# Autodesk Inventor assembly: Magnet
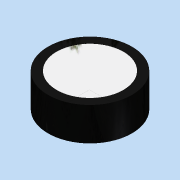
[picture p0: Inventor's stored thumbnail of the model, 180x180]
Saved by Autodesk Inventor 2015 (Build 190159000, 159)
## iProperties
Created: 2015-11-09
Part Number: Magnet
Document SubType Name: Assembly
Designer: Raphael
Author: Raphael
## Documents named in this file (3)
- \\psf\Home\Documents\electric-skateboard\CAD\Magnet.iam
- \\psf\Home\Documents\electric-skateboard\CAD\MagnetHolder.ipt
- \\psf\Home\Documents\electric-skateboard\CAD\Magnet.ipt
## Components (2 placed, 2 different names)
1. MagnetHolder:1 — Mate:1, Flush:1
2. Magnet:1 — Mate:1, Flush:1
## Relationships (2: Mate 1, Flush 1)
- Mate:1: MagnetHolder:1 ↔ Magnet:1
- Flush:1: MagnetHolder:1 ↔ Magnet:1
